# Autodesk Inventor assembly: Tuer
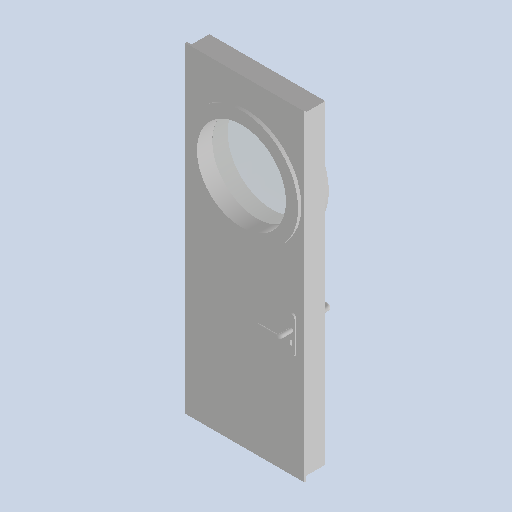
[picture p0: Inventor's stored thumbnail of the model, 512x512]
Saved by Autodesk Inventor 2025.1 (Build 291241000, 241)
## iProperties
Created: 2024-08-07
Part Number: Tuer
Document SubType Name: Assembly
Designer: ffogue
Author: ffogue
## Documents named in this file (6)
- C:\Users\ffogue\Documents\Inventor\BrandschutzTuer\Tuer.iam
- C:\Users\ffogue\Documents\Inventor\BrandschutzTuer\Rahmen.ipt
- C:\Users\ffogue\Documents\Inventor\BrandschutzTuer\Schutz.ipt
- C:\Users\ffogue\Documents\Inventor\BrandschutzTuer\garnitur_lang.ipt
- C:\Users\ffogue\Documents\Inventor\BrandschutzTuer\garnitur_lang_links.ipt
- C:\Users\ffogue\Documents\Inventor\BrandschutzTuer\glassMitSchutz.iam
## Components (5 placed, 5 different names)
1. Rahmen:1 — Flush:2, Flush:3, Flush:4, Mate:1, Mate:2, Insert:1
2. Schutz:1 — Flush:2, Flush:3, Flush:4, Mate:3, Mate:4, Insert:2, Insert:3
3. garnitur_lang:2 — Mate:1, Mate:2, Insert:1
4. garnitur_lang_links:1 — Mate:3, Mate:4, Insert:2
5. glassMitSchutz:1 [sub-assembly] — Insert:3
## Relationships (10: Mate 4, Flush 3, Insert 3)
- Flush:2 (9.5 mm): Rahmen:1 ↔ Schutz:1
- Flush:3 (19 mm): Rahmen:1 ↔ Schutz:1
- Flush:4 (-65 mm): Rahmen:1 ↔ Schutz:1
- Mate:1: Rahmen:1 ↔ garnitur_lang:2
- Mate:2: Rahmen:1 ↔ garnitur_lang:2
- Insert:1: Rahmen:1 ↔ garnitur_lang:2
- Mate:3: Schutz:1 ↔ garnitur_lang_links:1
- Mate:4: Schutz:1 ↔ garnitur_lang_links:1
- Insert:2: Schutz:1 ↔ garnitur_lang_links:1
- Insert:3: Schutz:1 ↔ glassMitSchutz:1
